# Autodesk Inventor assembly: ASSEMBLY_Main
(part 4 of 4)
- Mate:456: 3DP_PLA_Controller_Case_Fan_Grill:1 ↔ DIN 125-1 A A 4,3:7
- Mate:457: 3DP_PLA_Controller_Case_Fan_Grill:1 ↔ DIN 125-1 A A 4,3:8
- Mate:458: 3DP_PLA_Controller_Case_Fan_Grill:1 ↔ DIN 125-1 A A 4,3:8
- Mate:459: 3DP_PLA_Controller_Case_Fan_Grill:1 ↔ DIN 125-1 A A 4,3:9
- Mate:460: 3DP_PLA_Controller_Case_Fan_Grill:1 ↔ DIN 125-1 A A 4,3:9
- Insert:93: DIN 912 - replaced by DIN EN ISO 4762 M4 x 40:1 ↔ DIN 125-1 A A 4,3:5
- Insert:94: DIN 912 - replaced by DIN EN ISO 4762 M4 x 40:2 ↔ DIN 125-1 A A 4,3:7
- Insert:95: DIN 912 - replaced by DIN EN ISO 4762 M4 x 40:3 ↔ DIN 125-1 A A 4,3:8
- Insert:96: DIN 912 - replaced by DIN EN ISO 4762 M4 x 40:4 ↔ DIN 125-1 A A 4,3:9
- Mate:461: 3DP_PLA_Controller_Case_Fan_Grill:1 ↔ DIN 125-1 A A 4,3:6
- Mate:462: 3DP_PLA_Controller_Case_Top:1 ↔ DIN 125-1 A A 4,3:6
- Mate:463: 3DP_PLA_Controller_Case_Fan_Grill:1 ↔ DIN 125-1 A A 4,3:10
- Mate:464: 3DP_PLA_Controller_Case_Top:1 ↔ DIN 125-1 A A 4,3:10
- Mate:465: 3DP_PLA_Controller_Case_Fan_Grill:1 ↔ DIN 125-1 A A 4,3:11
- Mate:466: 3DP_PLA_Controller_Case_Top:1 ↔ DIN 125-1 A A 4,3:11
- Mate:467: 3DP_PLA_Controller_Case_Fan_Grill:1 ↔ DIN 125-1 A A 4,3:12
- Mate:468: 3DP_PLA_Controller_Case_Top:1 ↔ DIN 125-1 A A 4,3:12
- Insert:97: DIN 934 - replaced by DIN EN 24032/28673/28674 M4:3 ↔ DIN 125-1 A A 4,3:6
- Insert:98: DIN 934 - replaced by DIN EN 24032/28673/28674 M4:4 ↔ DIN 125-1 A A 4,3:10
- Insert:99: DIN 934 - replaced by DIN EN 24032/28673/28674 M4:5 ↔ DIN 125-1 A A 4,3:11
- Insert:100: DIN 934 - replaced by DIN EN 24032/28673/28674 M4:6 ↔ DIN 125-1 A A 4,3:12
- Mate:469: LC_ALU_4mm_Z_Axis_Motor_Mount:2 ↔ DIN 125-1 A A 5,3:56
- Mate:470: LC_ALU_4mm_Z_Axis_Motor_Mount:2 ↔ DIN 125-1 A A 5,3:56
- Mate:471: LC_ALU_4mm_Z_Axis_Motor_Mount:1 ↔ DIN 125-1 A A 5,3:55
- Mate:472: LC_ALU_4mm_Z_Axis_Motor_Mount:2 ↔ DIN 125-1 A A 5,3:55
- Insert:101: DIN 912 - replaced by DIN EN ISO 4762 M5 x 10:4 ↔ DIN 125-1 A A 5,3:56
- Insert:102: DIN 912 - replaced by DIN EN ISO 4762 M5 x 10:3 ↔ DIN 125-1 A A 5,3:55
- Mate:473: COTS_GENERIC_20x20mm_Angle_Bracket:5 ↔ DIN 125-1 A A 5,3:54
- Mate:474: COTS_GENERIC_20x20mm_Angle_Bracket:5 ↔ DIN 125-1 A A 5,3:54
- Mate:475: COTS_GENERIC_20x20mm_Angle_Bracket:2 ↔ DIN 125-1 A A 5,3:53
- Mate:476: COTS_GENERIC_20x20mm_Angle_Bracket:5 ↔ DIN 125-1 A A 5,3:53
- Insert:103: DIN 912 - replaced by DIN EN ISO 4762 M5 x 12:6 ↔ DIN 125-1 A A 5,3:54
- Insert:104: DIN 912 - replaced by DIN EN ISO 4762 M5 x 12:5 ↔ DIN 125-1 A A 5,3:53
- Mate:477: COTS_GENERIC_20x20mm_Angle_Bracket:8 ↔ DIN 125-1 A A 5,3:49
- Mate:478: COTS_GENERIC_20x20mm_Angle_Bracket:8 ↔ DIN 125-1 A A 5,3:49
- Mate:479: COTS_GENERIC_20x20mm_Angle_Bracket:3 ↔ DIN 125-1 A A 5,3:50
- Mate:480: COTS_GENERIC_20x20mm_Angle_Bracket:8 ↔ DIN 125-1 A A 5,3:50
- Insert:105: DIN 912 - replaced by DIN EN ISO 4762 M5 x 10:1 ↔ DIN 125-1 A A 5,3:49
- Insert:106: DIN 912 - replaced by DIN EN ISO 4762 M5 x 10:2 ↔ DIN 125-1 A A 5,3:50
- Mate:481: COTS_GENERIC_20x20mm_Angle_Bracket:5 ↔ DIN 125-1 A A 5,3:51
- Mate:482: COTS_GENERIC_20x20mm_Angle_Bracket:5 ↔ DIN 125-1 A A 5,3:51
- Mate:483: COTS_GENERIC_20x20mm_Angle_Bracket:2 ↔ DIN 125-1 A A 5,3:52
- Mate:484: COTS_GENERIC_20x20mm_Angle_Bracket:5 ↔ DIN 125-1 A A 5,3:52
- Insert:107: DIN 125-1 A A 5,3:51 ↔ DIN 912 - replaced by DIN EN ISO 4762 M5 x 10:5
- Insert:108: DIN 912 - replaced by DIN EN ISO 4762 M5 x 10:6 ↔ DIN 125-1 A A 5,3:52
- Mate:485: COTS_GENERIC_20x20mm_Angle_Bracket:8 ↔ DIN 125-1 A A 5,3:57
- Mate:486: COTS_GENERIC_20x20mm_Angle_Bracket:8 ↔ DIN 125-1 A A 5,3:57
- Mate:487: COTS_GENERIC_20x20mm_Angle_Bracket:3 ↔ DIN 125-1 A A 5,3:58
- Mate:488: COTS_GENERIC_20x20mm_Angle_Bracket:8 ↔ DIN 125-1 A A 5,3:58
- Insert:109: DIN 912 - replaced by DIN EN ISO 4762 M5 x 10:7 ↔ DIN 125-1 A A 5,3:57
- Insert:110: DIN 912 - replaced by DIN EN ISO 4762 M5 x 10:8 ↔ DIN 125-1 A A 5,3:58
- Mate:489: COTS_GENERIC_SK12_Linear_Rail_Mount:2 ↔ DIN 125-1 A A 5,3:59
- Mate:490: COTS_GENERIC_SK12_Linear_Rail_Mount:2 ↔ DIN 125-1 A A 5,3:59
- Mate:491: COTS_GENERIC_SK12_Linear_Rail_Mount:2 ↔ DIN 125-1 A A 5,3:60
- Mate:492: COTS_GENERIC_SK12_Linear_Rail_Mount:2 ↔ DIN 125-1 A A 5,3:60
- Insert:111: DIN 912 - replaced by DIN EN ISO 4762 M5 x 12:7 ↔ DIN 125-1 A A 5,3:59
- Insert:112: DIN 912 - replaced by DIN EN ISO 4762 M5 x 12:8 ↔ DIN 125-1 A A 5,3:60
- Mate:493: COTS_GENERIC_SK12_Linear_Rail_Mount:1 ↔ DIN 125-1 A A 5,3:61
- Mate:494: COTS_GENERIC_SK12_Linear_Rail_Mount:1 ↔ DIN 125-1 A A 5,3:61
- Mate:495: COTS_GENERIC_SK12_Linear_Rail_Mount:1 ↔ DIN 125-1 A A 5,3:62
- Mate:496: COTS_GENERIC_SK12_Linear_Rail_Mount:1 ↔ DIN 125-1 A A 5,3:62
- Insert:113: DIN 912 - replaced by DIN EN ISO 4762 M5 x 12:9 ↔ DIN 125-1 A A 5,3:61
- Insert:114: DIN 912 - replaced by DIN EN ISO 4762 M5 x 12:10 ↔ DIN 125-1 A A 5,3:62
- Mate:497: COTS_GENERIC_20x20mm_Angle_Bracket:6 ↔ DIN 125-1 A A 5,3:63
- Mate:498: COTS_GENERIC_20x20mm_Angle_Bracket:6 ↔ DIN 125-1 A A 5,3:63
- Mate:499: COTS_GENERIC_20x20mm_Angle_Bracket:1 ↔ DIN 125-1 A A 5,3:64
- Mate:500: COTS_GENERIC_20x20mm_Angle_Bracket:6 ↔ DIN 125-1 A A 5,3:64
- Insert:115: DIN 912 - replaced by DIN EN ISO 4762 M5 x 10:9 ↔ DIN 125-1 A A 5,3:63
- Insert:116: DIN 912 - replaced by DIN EN ISO 4762 M5 x 10:10 ↔ DIN 125-1 A A 5,3:64
- Mate:501: COTS_GENERIC_20x20mm_Angle_Bracket:4 ↔ DIN 125-1 A A 5,3:65
- Mate:502: COTS_GENERIC_20x20mm_Angle_Bracket:4 ↔ DIN 125-1 A A 5,3:65
- Mate:503: COTS_GENERIC_20x20mm_Angle_Bracket:7 ↔ DIN 125-1 A A 5,3:66
- Mate:504: COTS_GENERIC_20x20mm_Angle_Bracket:4 ↔ DIN 125-1 A A 5,3:66
- Insert:117: DIN 912 - replaced by DIN EN ISO 4762 M5 x 10:11 ↔ DIN 125-1 A A 5,3:65
- Insert:118: DIN 912 - replaced by DIN EN ISO 4762 M5 x 10:12 ↔ DIN 125-1 A A 5,3:66
- Mate:505: 3DP_PLA_Controller_Case_Top:1 ↔ DIN 125-1 A A 4,3:13
- Mate:506: 3DP_PLA_Controller_Case_Top:1 ↔ DIN 125-1 A A 4,3:13
- Mate:507: 3DP_PLA_Controller_Case_Top:1 ↔ DIN 125-1 A A 4,3:14
- Mate:508: 3DP_PLA_Controller_Case_Top:1 ↔ DIN 125-1 A A 4,3:14
- Mate:509: 3DP_PLA_Controller_Case_Top:1 ↔ DIN 125-1 A A 4,3:15
- Mate:510: 3DP_PLA_Controller_Case_Top:1 ↔ DIN 125-1 A A 4,3:15
- Mate:511: 3DP_PLA_Controller_Case_Top:1 ↔ DIN 125-1 A A 4,3:16
- Mate:512: 3DP_PLA_Controller_Case_Top:1 ↔ DIN 125-1 A A 4,3:16
- Insert:119: DIN 912 - replaced by DIN EN ISO 4762 M4 x 8:1 ↔ DIN 125-1 A A 4,3:13
- Insert:120: DIN 912 - replaced by DIN EN ISO 4762 M4 x 8:2 ↔ DIN 125-1 A A 4,3:14
- Insert:121: DIN 912 - replaced by DIN EN ISO 4762 M4 x 8:3 ↔ DIN 125-1 A A 4,3:15
- Insert:122: DIN 912 - replaced by DIN EN ISO 4762 M4 x 8:4 ↔ DIN 125-1 A A 4,3:16
- Mate:513: 3DP_PLA_Controller_Case_Bottom:1 ↔ DIN 125-1 A A 4,3:17
- Mate:514: 3DP_PLA_Controller_Case_Bottom:1 ↔ DIN 125-1 A A 4,3:17
- Mate:515: 3DP_PLA_Controller_Case_Bottom:1 ↔ DIN 125-1 A A 4,3:18
- Mate:516: 3DP_PLA_Controller_Case_Bottom:1 ↔ DIN 125-1 A A 4,3:18
- Mate:517: 3DP_PLA_Controller_Case_Bottom:1 ↔ DIN 125-1 A A 4,3:19
- Mate:518: 3DP_PLA_Controller_Case_Bottom:1 ↔ DIN 125-1 A A 4,3:19
- Mate:519: 3DP_PLA_Controller_Case_Bottom:1 ↔ DIN 125-1 A A 4,3:20
- Mate:520: 3DP_PLA_Controller_Case_Bottom:1 ↔ DIN 125-1 A A 4,3:20
- Insert:123: DIN 912 - replaced by DIN EN ISO 4762 M4 x 10:1 ↔ DIN 125-1 A A 4,3:17
- Insert:124: DIN 912 - replaced by DIN EN ISO 4762 M4 x 10:2 ↔ DIN 125-1 A A 4,3:18
- Insert:125: DIN 912 - replaced by DIN EN ISO 4762 M4 x 10:3 ↔ DIN 125-1 A A 4,3:19
- Insert:126: DIN 912 - replaced by DIN EN ISO 4762 M4 x 10:4 ↔ DIN 125-1 A A 4,3:20
- Mate:521: COTS_GENERIC_20x20mm_Angle_Bracket:1 ↔ DIN 125-1 A A 5,3:67
- Mate:522: COTS_GENERIC_20x20mm_Angle_Bracket:1 ↔ DIN 125-1 A A 5,3:67
- Mate:523: COTS_GENERIC_20x20mm_Angle_Bracket:4 ↔ DIN 125-1 A A 5,3:68
- Mate:524: COTS_GENERIC_20x20mm_Angle_Bracket:1 ↔ DIN 125-1 A A 5,3:68
- Insert:127: DIN 912 - replaced by DIN EN ISO 4762 M5 x 10:13 ↔ DIN 125-1 A A 5,3:67
- Insert:128: DIN 912 - replaced by DIN EN ISO 4762 M5 x 10:14 ↔ DIN 125-1 A A 5,3:68
- Mate:525: COTS_GENERIC_20x20mm_Angle_Bracket:6 ↔ DIN 125-1 A A 5,3:69
- Mate:526: COTS_GENERIC_20x20mm_Angle_Bracket:6 ↔ DIN 125-1 A A 5,3:69
- Mate:527: COTS_GENERIC_20x20mm_Angle_Bracket:7 ↔ DIN 125-1 A A 5,3:70
- Mate:528: COTS_GENERIC_20x20mm_Angle_Bracket:6 ↔ DIN 125-1 A A 5,3:70
- Insert:129: DIN 912 - replaced by DIN EN ISO 4762 M5 x 10:15 ↔ DIN 125-1 A A 5,3:69
- Insert:130: DIN 912 - replaced by DIN EN ISO 4762 M5 x 10:16 ↔ DIN 125-1 A A 5,3:70
- Mate:529: COTS_GENERIC_SHF10_Linear_Rail_Mount:4 ↔ DIN 125-1 A A 5,3:71
- Mate:530: COTS_GENERIC_SHF10_Linear_Rail_Mount:4 ↔ DIN 125-1 A A 5,3:71
- Mate:531: COTS_GENERIC_SHF10_Linear_Rail_Mount:4 ↔ DIN 125-1 A A 5,3:72
- Mate:532: COTS_GENERIC_SHF10_Linear_Rail_Mount:4 ↔ DIN 125-1 A A 5,3:72
- Mate:533: COTS_GENERIC_SHF10_Linear_Rail_Mount:3 ↔ DIN 125-1 A A 5,3:73
- Mate:534: COTS_GENERIC_SHF10_Linear_Rail_Mount:4 ↔ DIN 125-1 A A 5,3:73
- Mate:535: COTS_GENERIC_SHF10_Linear_Rail_Mount:3 ↔ DIN 125-1 A A 5,3:74
- Mate:536: COTS_GENERIC_SHF10_Linear_Rail_Mount:4 ↔ DIN 125-1 A A 5,3:74
- Insert:131: DIN 912 - replaced by DIN EN ISO 4762 M5 x 10:17 ↔ DIN 125-1 A A 5,3:71
- Insert:132: DIN 912 - replaced by DIN EN ISO 4762 M5 x 10:18 ↔ DIN 125-1 A A 5,3:72
- Insert:133: DIN 912 - replaced by DIN EN ISO 4762 M5 x 10:19 ↔ DIN 125-1 A A 5,3:73
- Insert:134: DIN 912 - replaced by DIN EN ISO 4762 M5 x 10:20 ↔ DIN 125-1 A A 5,3:74
- Mate:537: COTS_GENERIC_SHF10_Linear_Rail_Mount:2 ↔ DIN 125-1 A A 5,3:75
- Mate:538: COTS_GENERIC_SHF10_Linear_Rail_Mount:2 ↔ DIN 125-1 A A 5,3:75
- Mate:539: COTS_GENERIC_SHF10_Linear_Rail_Mount:2 ↔ DIN 125-1 A A 5,3:76
- Mate:540: COTS_GENERIC_SHF10_Linear_Rail_Mount:2 ↔ DIN 125-1 A A 5,3:76
- Mate:541: COTS_GENERIC_SHF10_Linear_Rail_Mount:1 ↔ DIN 125-1 A A 5,3:77
- Mate:542: COTS_GENERIC_SHF10_Linear_Rail_Mount:2 ↔ DIN 125-1 A A 5,3:77
- Mate:543: COTS_GENERIC_SHF10_Linear_Rail_Mount:1 ↔ DIN 125-1 A A 5,3:78
- Mate:544: COTS_GENERIC_SHF10_Linear_Rail_Mount:2 ↔ DIN 125-1 A A 5,3:78
- Insert:135: DIN 912 - replaced by DIN EN ISO 4762 M5 x 10:21 ↔ DIN 125-1 A A 5,3:75
- Insert:136: DIN 912 - replaced by DIN EN ISO 4762 M5 x 10:22 ↔ DIN 125-1 A A 5,3:76
- Insert:137: DIN 912 - replaced by DIN EN ISO 4762 M5 x 10:23 ↔ DIN 125-1 A A 5,3:77
- Insert:138: DIN 912 - replaced by DIN EN ISO 4762 M5 x 10:24 ↔ DIN 125-1 A A 5,3:78
- Mate:545: CNCM_ALU_3mm_Y_Axis_Idler_Stiffener_Side:2 ↔ DIN 125-1 A A 5,3:79
- Mate:546: CNCM_ALU_3mm_Y_Axis_Idler_Stiffener_Side:2 ↔ DIN 125-1 A A 5,3:79
- Mate:547: CNCM_ALU_3mm_Y_Axis_Idler_Stiffener_Side:1 ↔ DIN 125-1 A A 5,3:80
- Mate:548: CNCM_ALU_3mm_Y_Axis_Idler_Stiffener_Side:2 ↔ DIN 125-1 A A 5,3:80
- Insert:139: DIN 912 - replaced by DIN EN ISO 4762 M5 x 8:21 ↔ DIN 125-1 A A 5,3:79
- Insert:140: DIN 912 - replaced by DIN EN ISO 4762 M5 x 8:22 ↔ DIN 125-1 A A 5,3:80
- Mate:549: LCBN_ALU_3mm_Y_Axis_Idler_Stiffener_Top:1 ↔ DIN 125-1 A A 5,3:81
- Mate:550: LCBN_ALU_3mm_Y_Axis_Idler_Stiffener_Top:1 ↔ DIN 125-1 A A 5,3:81
- Insert:141: DIN 912 - replaced by DIN EN ISO 4762 M5 x 30:13 ↔ DIN 125-1 A A 5,3:81
- Mate:551: CNCM_ALU_3mm_Y_Axis_Idler_Stiffener_Side:2 ↔ DIN 125-1 A A 3,2:44
- Mate:552: CNCM_ALU_3mm_Y_Axis_Idler_Stiffener_Side:2 ↔ DIN 125-1 A A 3,2:44
- Mate:553: CNCM_ALU_3mm_Y_Axis_Idler_Stiffener_Side:2 ↔ DIN 125-1 A A 3,2:46
- Mate:554: CNCM_ALU_3mm_Y_Axis_Idler_Stiffener_Side:2 ↔ DIN 125-1 A A 3,2:46
- Insert:142: DIN 912 - replaced by DIN EN ISO 4762 M3 x 10:1 ↔ DIN 125-1 A A 3,2:44
- Insert:143: DIN 912 - replaced by DIN EN ISO 4762 M3 x 10:2 ↔ DIN 125-1 A A 3,2:46
- Mate:555: CNCM_ALU_3mm_Y_Axis_Idler_Stiffener_Side:2 ↔ DIN 125-1 A A 3,2:45
- Mate:556: LCBN_ALU_3mm_Y_Axis_Idler_Stiffener_Top:1 ↔ DIN 125-1 A A 3,2:45
- Mate:557: CNCM_ALU_3mm_Y_Axis_Idler_Stiffener_Side:2 ↔ DIN 125-1 A A 3,2:47
- Mate:558: LCBN_ALU_3mm_Y_Axis_Idler_Stiffener_Top:1 ↔ DIN 125-1 A A 3,2:47
- Insert:144: DIN 934 - replaced by DIN EN 24032/28673/28674 M3:12 ↔ DIN 125-1 A A 3,2:45
- Insert:145: DIN 934 - replaced by DIN EN 24032/28673/28674 M3:13 ↔ DIN 125-1 A A 3,2:47
- Mate:559: CNCM_ALU_3mm_Y_Axis_Idler_Stiffener_Side:1 ↔ DIN 125-1 A A 3,2:48
- Mate:560: CNCM_ALU_3mm_Y_Axis_Idler_Stiffener_Side:1 ↔ DIN 125-1 A A 3,2:48
- Mate:561: CNCM_ALU_3mm_Y_Axis_Idler_Stiffener_Side:1 ↔ DIN 125-1 A A 3,2:50
- Mate:562: CNCM_ALU_3mm_Y_Axis_Idler_Stiffener_Side:1 ↔ DIN 125-1 A A 3,2:50
- Insert:146: DIN 912 - replaced by DIN EN ISO 4762 M3 x 10:3 ↔ DIN 125-1 A A 3,2:48
- Insert:147: DIN 912 - replaced by DIN EN ISO 4762 M3 x 10:4 ↔ DIN 125-1 A A 3,2:50
- Mate:563: CNCM_ALU_3mm_Y_Axis_Idler_Stiffener_Side:1 ↔ DIN 125-1 A A 3,2:49
- Mate:564: LCBN_ALU_3mm_Y_Axis_Idler_Stiffener_Top:1 ↔ DIN 125-1 A A 3,2:49
- Mate:565: CNCM_ALU_3mm_Y_Axis_Idler_Stiffener_Side:1 ↔ DIN 125-1 A A 3,2:51
- Mate:566: LCBN_ALU_3mm_Y_Axis_Idler_Stiffener_Top:1 ↔ DIN 125-1 A A 3,2:51
- Insert:148: DIN 934 - replaced by DIN EN 24032/28673/28674 M3:14 ↔ DIN 125-1 A A 3,2:49
- Insert:149: DIN 934 - replaced by DIN EN 24032/28673/28674 M3:15 ↔ DIN 125-1 A A 3,2:51
- Mate:567: LCBN_ALU_2mm_Y_Axis_Motor_Mount:1 ↔ DIN 125-1 A A 3,2:52
- Mate:568: LCBN_ALU_2mm_Y_Axis_Motor_Mount:1 ↔ DIN 125-1 A A 3,2:52
- Mate:569: LCBN_ALU_2mm_Y_Axis_Motor_Mount:1 ↔ DIN 125-1 A A 3,2:54
- Mate:570: LCBN_ALU_2mm_Y_Axis_Motor_Mount:1 ↔ DIN 125-1 A A 3,2:54
- Mate:571: LCBN_ALU_2mm_Y_Axis_Motor_Mount:1 ↔ DIN 125-1 A A 3,2:55
- Mate:572: LCBN_ALU_2mm_Y_Axis_Motor_Mount:1 ↔ DIN 125-1 A A 3,2:55
- Mate:573: LCBN_ALU_2mm_Y_Axis_Motor_Mount:1 ↔ DIN 125-1 A A 3,2:56
- Mate:574: LCBN_ALU_2mm_Y_Axis_Motor_Mount:1 ↔ DIN 125-1 A A 3,2:56
- Insert:150: DIN 912 - replaced by DIN EN ISO 4762 M3 x 16:5 ↔ DIN 125-1 A A 3,2:52
- Insert:151: DIN 912 - replaced by DIN EN ISO 4762 M3 x 16:6 ↔ DIN 125-1 A A 3,2:54
- Insert:152: DIN 912 - replaced by DIN EN ISO 4762 M3 x 16:7 ↔ DIN 125-1 A A 3,2:55
- Insert:153: DIN 912 - replaced by DIN EN ISO 4762 M3 x 16:8 ↔ DIN 125-1 A A 3,2:56
- Mate:575: LCBN_ALU_2mm_Y_Axis_Motor_Mount:1 ↔ DIN 125-1 A A 3,2:53
- Mate:576: COTS_GENERIC_NEMA23_Stepper_Motor:1 ↔ DIN 125-1 A A 3,2:53
- Mate:577: LCBN_ALU_2mm_Y_Axis_Motor_Mount:1 ↔ DIN 125-1 A A 3,2:57
- Mate:578: COTS_GENERIC_NEMA23_Stepper_Motor:1 ↔ DIN 125-1 A A 3,2:57
- Mate:579: LCBN_ALU_2mm_Y_Axis_Motor_Mount:1 ↔ DIN 125-1 A A 3,2:58
- Mate:580: COTS_GENERIC_NEMA23_Stepper_Motor:1 ↔ DIN 125-1 A A 3,2:58
- Mate:581: LCBN_ALU_2mm_Y_Axis_Motor_Mount:1 ↔ DIN 125-1 A A 3,2:59
- Mate:582: COTS_GENERIC_NEMA23_Stepper_Motor:1 ↔ DIN 125-1 A A 3,2:59
- Insert:154: DIN 934 - replaced by DIN EN 24032/28673/28674 M3:16 ↔ DIN 125-1 A A 3,2:53
- Insert:155: DIN 125-1 A A 3,2:57 ↔ DIN 934 - replaced by DIN EN 24032/28673/28674 M3:17
- Insert:156: DIN 125-1 A A 3,2:58 ↔ DIN 934 - replaced by DIN EN 24032/28673/28674 M3:18
- Insert:157: DIN 125-1 A A 3,2:59 ↔ DIN 934 - replaced by DIN EN 24032/28673/28674 M3:19
- Mate:583: LCBN_ALU_2mm_Y_Axis_Motor_Mount:1 ↔ DIN 125-1 A A 5,3:82
- Mate:584: LCBN_ALU_2mm_Y_Axis_Motor_Mount:1 ↔ DIN 125-1 A A 5,3:82
- Mate:585: LCBN_ALU_2mm_Y_Axis_Motor_Mount:1 ↔ DIN 125-1 A A 5,3:83
- Mate:586: LCBN_ALU_2mm_Y_Axis_Motor_Mount:1 ↔ DIN 125-1 A A 5,3:83
- Insert:158: DIN 912 - replaced by DIN EN ISO 4762 M5 x 8:23 ↔ DIN 125-1 A A 5,3:82
- Insert:159: DIN 912 - replaced by DIN EN ISO 4762 M5 x 8:24 ↔ DIN 125-1 A A 5,3:83
- Mate:587: LCBN_ALU_2mm_Y_Axis_Motor_Mount:1 ↔ DIN 125-1 A A 5,3:84
- Mate:588: LCBN_ALU_2mm_Y_Axis_Motor_Mount:1 ↔ DIN 125-1 A A 5,3:84
- Mate:589: LCBN_ALU_2mm_Y_Axis_Motor_Mount:1 ↔ DIN 125-1 A A 5,3:85
- Mate:590: LCBN_ALU_2mm_Y_Axis_Motor_Mount:1 ↔ DIN 125-1 A A 5,3:85
- Insert:160: DIN 912 - replaced by DIN EN ISO 4762 M5 x 12:11 ↔ DIN 125-1 A A 5,3:84
- Insert:161: DIN 912 - replaced by DIN EN ISO 4762 M5 x 12:12 ↔ DIN 125-1 A A 5,3:85
- Mate:591: 3DP_ABS_Y_Axis_Endstop_Mount:1 ↔ DIN 125-1 A A 5,3:86
- Mate:592: 3DP_ABS_Y_Axis_Endstop_Mount:1 ↔ DIN 125-1 A A 5,3:86
- Insert:162: DIN 912 - replaced by DIN EN ISO 4762 M5 x 8:25 ↔ DIN 125-1 A A 5,3:86
- Mate:593: 3DP_ABS_Feet:3 ↔ DIN 125-1 A A 5,3:87
- Mate:594: 3DP_ABS_Feet:3 ↔ DIN 125-1 A A 5,3:87
- Mate:595: 3DP_ABS_Feet_MIR:1 ↔ DIN 125-1 A A 5,3:88
- Mate:596: 3DP_ABS_Feet:3 ↔ DIN 125-1 A A 5,3:88
- Mate:597: 3DP_ABS_Feet:1 ↔ DIN 125-1 A A 5,3:89
- Mate:598: 3DP_ABS_Feet:3 ↔ DIN 125-1 A A 5,3:89
- Mate:599: 3DP_ABS_Feet_MIR:2 ↔ DIN 125-1 A A 5,3:90
- Mate:600: 3DP_ABS_Feet:3 ↔ DIN 125-1 A A 5,3:90
- Insert:163: DIN 912 - replaced by DIN EN ISO 4762 M5 x 10:25 ↔ DIN 125-1 A A 5,3:87
- Insert:164: DIN 912 - replaced by DIN EN ISO 4762 M5 x 10:26 ↔ DIN 125-1 A A 5,3:88
- Insert:165: DIN 912 - replaced by DIN EN ISO 4762 M5 x 10:27 ↔ DIN 125-1 A A 5,3:89
- Insert:166: DIN 912 - replaced by DIN EN ISO 4762 M5 x 10:28 ↔ DIN 125-1 A A 5,3:90
- Mate:601: 3DP_ABS_Feet_MIR:1 ↔ DIN 125-1 A A 5,3:91
- Mate:602: 3DP_ABS_Feet_MIR:1 ↔ DIN 125-1 A A 5,3:91
- Mate:603: 3DP_ABS_Feet:1 ↔ DIN 125-1 A A 5,3:92
- Mate:604: 3DP_ABS_Feet_MIR:1 ↔ DIN 125-1 A A 5,3:92
- Mate:605: 3DP_ABS_Feet_MIR:2 ↔ DIN 125-1 A A 5,3:93
- Mate:606: 3DP_ABS_Feet_MIR:1 ↔ DIN 125-1 A A 5,3:93
- Mate:607: 3DP_ABS_Feet:3 ↔ DIN 125-1 A A 5,3:94
- Mate:608: 3DP_ABS_Feet_MIR:1 ↔ DIN 125-1 A A 5,3:94
- Insert:167: DIN 912 - replaced by DIN EN ISO 4762 M5 x 10:29 ↔ DIN 125-1 A A 5,3:91
- Insert:168: DIN 912 - replaced by DIN EN ISO 4762 M5 x 10:30 ↔ DIN 125-1 A A 5,3:92
- Insert:169: DIN 912 - replaced by DIN EN ISO 4762 M5 x 10:31 ↔ DIN 125-1 A A 5,3:93
- Insert:170: DIN 912 - replaced by DIN EN ISO 4762 M5 x 10:32 ↔ DIN 125-1 A A 5,3:94
- Mate:609: LCBN_STEEL_3mm_Y_Axis_Heatbed_Baseplate:1 ↔ DIN 912 - replaced by DIN EN ISO 4762 M3 x 30:1
- Mate:610: LCBN_STEEL_3mm_Y_Axis_Heatbed_Baseplate:1 ↔ DIN 912 - replaced by DIN EN ISO 4762 M3 x 30:1
- Mate:611: 3DP_ABS_Y_Axis_Linear_Bearing_Mount_Bottom:4 ↔ DIN 912 - replaced by DIN EN ISO 4762 M3 x 30:2
- Mate:612: LCBN_STEEL_3mm_Y_Axis_Heatbed_Baseplate:1 ↔ DIN 912 - replaced by DIN EN ISO 4762 M3 x 30:2
- Mate:613: 3DP_ABS_Y_Axis_Linear_Bearing_Mount_Bottom:2 ↔ DIN 912 - replaced by DIN EN ISO 4762 M3 x 30:3
- Mate:614: LCBN_STEEL_3mm_Y_Axis_Heatbed_Baseplate:1 ↔ DIN 912 - replaced by DIN EN ISO 4762 M3 x 30:3
- Mate:615: 3DP_ABS_Y_Axis_Linear_Bearing_Mount_Bottom:2 ↔ DIN 912 - replaced by DIN EN ISO 4762 M3 x 30:4
- Mate:616: LCBN_STEEL_3mm_Y_Axis_Heatbed_Baseplate:1 ↔ DIN 912 - replaced by DIN EN ISO 4762 M3 x 30:4
- Mate:617: 3DP_ABS_Y_Axis_Linear_Bearing_Mount_Bottom:3 ↔ DIN 912 - replaced by DIN EN ISO 4762 M3 x 30:5
- Mate:618: LCBN_STEEL_3mm_Y_Axis_Heatbed_Baseplate:1 ↔ DIN 912 - replaced by DIN EN ISO 4762 M3 x 30:5
- Mate:619: 3DP_ABS_Y_Axis_Linear_Bearing_Mount_Bottom:3 ↔ DIN 912 - replaced by DIN EN ISO 4762 M3 x 30:6
- Mate:620: LCBN_STEEL_3mm_Y_Axis_Heatbed_Baseplate:1 ↔ DIN 912 - replaced by DIN EN ISO 4762 M3 x 30:6
- Mate:621: 3DP_ABS_Y_Axis_Linear_Bearing_Mount_Bottom:1 ↔ DIN 912 - replaced by DIN EN ISO 4762 M3 x 30:7
- Mate:622: LCBN_STEEL_3mm_Y_Axis_Heatbed_Baseplate:1 ↔ DIN 912 - replaced by DIN EN ISO 4762 M3 x 30:7
- Mate:623: 3DP_ABS_Y_Axis_Linear_Bearing_Mount_Bottom:1 ↔ DIN 912 - replaced by DIN EN ISO 4762 M3 x 30:8
- Mate:624: LCBN_STEEL_3mm_Y_Axis_Heatbed_Baseplate:1 ↔ DIN 912 - replaced by DIN EN ISO 4762 M3 x 30:8
- Mate:625: LCBN_STEEL_3mm_Y_Axis_Heatbed_Baseplate:1 ↔ DIN 934 - replaced by DIN EN 24032/28673/28674 M3:20
- Mate:626: 3DP_ABS_Y_Axis_Linear_Bearing_Mount_Bottom:4 ↔ DIN 934 - replaced by DIN EN 24032/28673/28674 M3:20
- Mate:627: 3DP_ABS_Y_Axis_Linear_Bearing_Mount_Bottom:4 ↔ DIN 934 - replaced by DIN EN 24032/28673/28674 M3:21
- Mate:628: 3DP_ABS_Y_Axis_Linear_Bearing_Mount_Bottom:4 ↔ DIN 934 - replaced by DIN EN 24032/28673/28674 M3:21
- Mate:629: 3DP_ABS_Y_Axis_Linear_Bearing_Mount_Bottom:2 ↔ DIN 934 - replaced by DIN EN 24032/28673/28674 M3:22
- Mate:630: 3DP_ABS_Y_Axis_Linear_Bearing_Mount_Bottom:4 ↔ DIN 934 - replaced by DIN EN 24032/28673/28674 M3:22
- Mate:631: 3DP_ABS_Y_Axis_Linear_Bearing_Mount_Bottom:2 ↔ DIN 934 - replaced by DIN EN 24032/28673/28674 M3:23
- Mate:632: 3DP_ABS_Y_Axis_Linear_Bearing_Mount_Bottom:4 ↔ DIN 934 - replaced by DIN EN 24032/28673/28674 M3:23
- Mate:633: 3DP_ABS_Y_Axis_Linear_Bearing_Mount_Bottom:3 ↔ DIN 934 - replaced by DIN EN 24032/28673/28674 M3:24
- Mate:634: 3DP_ABS_Y_Axis_Linear_Bearing_Mount_Bottom:4 ↔ DIN 934 - replaced by DIN EN 24032/28673/28674 M3:24
- Mate:635: 3DP_ABS_Y_Axis_Linear_Bearing_Mount_Bottom:3 ↔ DIN 934 - replaced by DIN EN 24032/28673/28674 M3:25
- Mate:636: 3DP_ABS_Y_Axis_Linear_Bearing_Mount_Bottom:4 ↔ DIN 934 - replaced by DIN EN 24032/28673/28674 M3:25
- Mate:637: 3DP_ABS_Y_Axis_Linear_Bearing_Mount_Bottom:1 ↔ DIN 934 - replaced by DIN EN 24032/28673/28674 M3:26
- Mate:638: 3DP_ABS_Y_Axis_Linear_Bearing_Mount_Bottom:4 ↔ DIN 934 - replaced by DIN EN 24032/28673/28674 M3:26
- Mate:639: 3DP_ABS_Y_Axis_Linear_Bearing_Mount_Bottom:1 ↔ DIN 934 - replaced by DIN EN 24032/28673/28674 M3:27
- Mate:640: 3DP_ABS_Y_Axis_Linear_Bearing_Mount_Bottom:4 ↔ DIN 934 - replaced by DIN EN 24032/28673/28674 M3:27
- Mate:641: CNCM_ALU_6mm_Heatbed:1 ↔ ISO 10642 M4x20:1
- Mate:642: CNCM_ALU_6mm_Heatbed:1 ↔ ISO 10642 M4x20:1
- Insert:171: LCBN_STEEL_3mm_Y_Axis_Heatbed_Baseplate:1 ↔ DIN 934 - replaced by DIN EN 24032/28673/28674 M4:7
- Insert:172: LCBN_STEEL_3mm_Y_Axis_Heatbed_Baseplate:1 ↔ DIN 934 - replaced by DIN EN 24032/28673/28674 M4:8
